# Autodesk Inventor assembly: RearUpperAArmandBracket
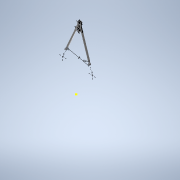
[picture p0: Inventor's stored thumbnail of the model, 180x180]
Saved by Autodesk Inventor 2021 (Build 250183000, 183)
## iProperties
Created: 2019-09-17
Part Number: RearUpperAArmandBracket
Document SubType Name: Assembly
Designer: beckerdj
Author: beckerdj
## Documents named in this file (11)
- C:\Users\cooks\Downloads\RearUpperAArmandBracket (1).iam
- C:\Users\cooks\Downloads\Weld Cup Model.ipt
- C:\Users\cooks\Downloads\UpperControlArmTubeF.ipt
- C:\Users\cooks\Downloads\Weldable Tube End.ipt
- C:\Users\cooks\Downloads\60645K131_STEEL BALL JOINT ROD END.ipt
- C:\Users\cooks\Downloads\63195K670_STEEL BALL JOINT SWIVEL BEARING.ipt
- C:\Users\cooks\Downloads\RIGHT BRACKET ARM FLAT (1).ipt
- C:\Users\cooks\Downloads\RIGHT BRACKET ARM FLAT (2).ipt
- C:\Users\cooks\Downloads\Bushings_MC_Mounting.ipt
- C:\Users\cooks\Downloads\FinalFrontLowerPlate.ipt
- C:\Users\cooks\Downloads\LowControlArmPlateTabF.ipt
## Components (15 placed, 10 different names)
1. Weld Cup Model:1 — Insert:5, Mate:10
2. UpperControlArmTubeF:1 — Insert:1, Mate:12
3. UpperControlArmTubeF:2 — Insert:2, Mate:11
4. Weldable Tube End:1 — Insert:2, Insert:4
5. Weldable Tube End:2 — Insert:1, Insert:3
6. 60645K131_STEEL BALL JOINT ROD END:1 — Insert:3, Mate:6, Mate:9
7. 60645K131_STEEL BALL JOINT ROD END:2 — Insert:4, Mate:7
8. 63195K670_STEEL BALL JOINT SWIVEL BEARING:1 — Insert:5
9. FinalFrontLowerPlate:1 — Mate:10, Mate:11, Mate:12, Mate:13, Mate:14
10. RIGHT BRACKET ARM FLAT (1):1 — Mate:6
11. RIGHT BRACKET ARM FLAT (2):1 — Mate:7, Mate:8
12. Bushings_MC_Mounting:1 — Mate:8
13. Bushings_MC_Mounting:2 — Mate:9
14. LowControlArmPlateTabF:1 — Mate:14, Flush:2
15. LowControlArmPlateTabF:2 — Mate:13, Flush:2
## Relationships (23: Mate 14, Insert 5, Flush 2, Tangent 2)
- Insert:1: UpperControlArmTubeF:1 ↔ Weldable Tube End:2
- Insert:2: UpperControlArmTubeF:2 ↔ Weldable Tube End:1
- Insert:3: Weldable Tube End:2 ↔ 60645K131_STEEL BALL JOINT ROD END:1
- Insert:4: Weldable Tube End:1 ↔ 60645K131_STEEL BALL JOINT ROD END:2
- Insert:5: Weld Cup Model:1 ↔ 63195K670_STEEL BALL JOINT SWIVEL BEARING:1
- [Mate]: Weld Cup Model:1 ↔ FinalFrontLowerPlate:1
- [Flush] (-4.7244 mm): Weld Cup Model:1 ↔ FinalFrontLowerPlate:1
- [Mate]: UpperControlArmTubeF:2 ↔ FinalFrontLowerPlate:1
- [Mate]: UpperControlArmTubeF:2 ↔ FinalFrontLowerPlate:1
- [Mate]: UpperControlArmTubeF:1 ↔ FinalFrontLowerPlate:1
- [Mate]: UpperControlArmTubeF:1 ↔ FinalFrontLowerPlate:1
- [Tangent] (0.762 mm): UpperControlArmTubeF:2 ↔ FinalFrontLowerPlate:1
- [Tangent] (0.762 mm): UpperControlArmTubeF:1 ↔ FinalFrontLowerPlate:1
- Mate:6: 60645K131_STEEL BALL JOINT ROD END:1 ↔ RIGHT BRACKET ARM FLAT (1):1
- Mate:7: 60645K131_STEEL BALL JOINT ROD END:2 ↔ RIGHT BRACKET ARM FLAT (2):1
- Mate:8: RIGHT BRACKET ARM FLAT (2):1 ↔ Bushings_MC_Mounting:1
- Mate:9: 60645K131_STEEL BALL JOINT ROD END:1 ↔ Bushings_MC_Mounting:2
- Mate:10: Weld Cup Model:1 ↔ FinalFrontLowerPlate:1
- Mate:11: UpperControlArmTubeF:2 ↔ FinalFrontLowerPlate:1
- Mate:12: UpperControlArmTubeF:1 ↔ FinalFrontLowerPlate:1
- Mate:13: FinalFrontLowerPlate:1 ↔ LowControlArmPlateTabF:2
- Mate:14: FinalFrontLowerPlate:1 ↔ LowControlArmPlateTabF:1
- Flush:2: LowControlArmPlateTabF:1 ↔ LowControlArmPlateTabF:2
